# Autodesk Inventor assembly: Robotunits GUS_4041 (75)
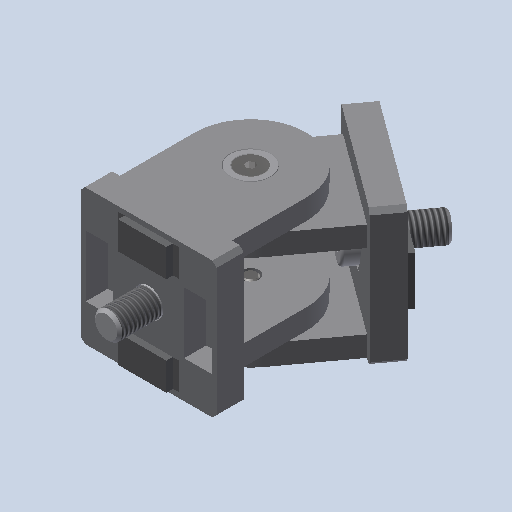
[picture p0: Inventor's stored thumbnail of the model, 512x512]
Saved by Autodesk Inventor 2023 (Build 270158000, 158)
## iProperties
Category: PARTsolutions
Company: ROBOTUNITS
Created: 2023-08-22
Part Number: Robotunits GUS_4041 (75)
Catalog Web Link: www.cadenas.de
Description: GUS 4_41-Elbow joint with clamp, kit
Vendor: ROBOTUNITS
Document SubType Name: Assembly
Designer: psAdmin
Manufacturer: ROBOTUNITS
Mass: 54.643 g
Surface Area: 289.943 cm^2
Volume: 52.1063 cm^3
Density: 1.04868 g/cm^3
PSOL_IDENT_0: {$CADENAS_DATA/23d-libs/robotunits/profil_und_verbindungstechnik/verbindungstechnik_raster_40/gus404
PSOL_IDENT_1: 1_asmtbl.prj},211 {VTYP=3D},{STYP=ASSTAB},{NB=Robotunits GUS_4041 (75)},{LINA=Robotunits GUS_4041},{
PSOL_IDENT_2: NN=GUS 4_41},{DATE=20.06.2022 09:55:41},{GEOMDATE=24.10.2014 07:53:29},{VERSION=},{LINEID=10},{WBVAR=
PSOL_IDENT_3: WINKEL},{WBNUMERIC=WINKEL}  {NB=Robotunits GUS_4041 (75)},{LINA=Robotunits GUS_4041},{KT=DUMMY},{ART
PSOL_IDENT_4: IKEL=GUS_4041},{WINKEL=75},{PPATH=parts/gus4041_sbl.prj},{FORM=1.000},{ROB=GUS4041},{ROBX=http://www
PSOL_IDENT_5: .robotunits.com/$CADENAS_LANGUAGE./Webshop/Verbindungstechnik/shopitem/gelenk-set/180/}
NB: Robotunits GUS_4041 (75)
NN: GUS 4_41
NT: Elbow joint with clamp, kit
NBSYN: Robotunits $ARTIKEL. ($WINKEL.)
LINA: Robotunits GUS_4041
CATALOG: Robotunits
ARTIKEL: GUS_4041
WINKEL: 75
ROB: GUS4041
SUPPLIER: ROBOTUNITS
ARTICLENO: Robotunits GUS_4041 (75)
BOMINFO: Robotunits GUS_4041
CREATOR: CADENAS GmbH
Title: Robotunits GUS_4041
Author: Cadenas PARTsolutions
Comments: Elbow joint with clamp, kit
## Documents named in this file (7)
- C:\work\robots\butler_2.0\body_model\parts\Elbow joint 40\Elbow joint 40.iam
- C:\work\robots\butler_2.0\body_model\parts\Elbow joint 40\Robotunits GUS_4040 75.ipt
- C:\work\robots\butler_2.0\body_model\parts\Elbow joint 40\GUS Zentriereinsatz.ipt
- C:\work\robots\butler_2.0\body_model\parts\Elbow joint 40\Robotunits IBS M8x16.ipt
- C:\work\robots\butler_2.0\body_model\parts\Elbow joint 40\Robotunits GUS_4040 -90.ipt
- C:\Users\chriboehm\Documents\Inventor\Content Center Files\R2023\en-US\DIN 7991(2)\DIN 7991 - M4x12.ipt
- C:\work\robots\butler_2.0\body_model\parts\Elbow joint 40\Washer.ipt
## Components (12 placed, 6 different names)
1. Robotunits GUS_4040 75:1 — Flush:1, Mate:7, Mate:10, Mate:13, Flush:4
2. GUS Zentriereinsatz:1
3. GUS Zentriereinsatz:2
4. Robotunits IBS M8x16:1
5. Robotunits GUS_4040 -90:1 — Mate:1, Mate:2, Mate:3, Mate:4, Mate:5, Mate:6, Flush:1, Mate:7, Mate:8, Mate:9, Mate:11, Mate:12, Flush:2
6. GUS Zentriereinsatz:3 — Mate:4, Mate:5, Mate:6
7. GUS Zentriereinsatz:4 — Mate:1, Mate:2, Mate:3
8. Robotunits IBS M8x16:2 — Mate:8, Mate:9
9. DIN 7991 M4x12:1 — Mate:10, Flush:5
10. DIN 7991 M4x12:2 — Mate:11, Flush:3
11. Washer:1 — Mate:12, Flush:2, Flush:3
12. Washer:2 — Mate:13, Flush:4, Flush:5
## Relationships (18: Mate 13, Flush 5)
- Mate:1: Robotunits GUS_4040 -90:1 ↔ GUS Zentriereinsatz:4
- Mate:2: Robotunits GUS_4040 -90:1 ↔ GUS Zentriereinsatz:4
- Mate:3: Robotunits GUS_4040 -90:1 ↔ GUS Zentriereinsatz:4
- Mate:4: Robotunits GUS_4040 -90:1 ↔ GUS Zentriereinsatz:3
- Mate:5: Robotunits GUS_4040 -90:1 ↔ GUS Zentriereinsatz:3
- Mate:6: Robotunits GUS_4040 -90:1 ↔ GUS Zentriereinsatz:3
- Flush:1: Robotunits GUS_4040 75:1 ↔ Robotunits GUS_4040 -90:1
- Mate:7: Robotunits GUS_4040 75:1 ↔ Robotunits GUS_4040 -90:1
- Mate:8: Robotunits GUS_4040 -90:1 ↔ Robotunits IBS M8x16:2
- Mate:9: Robotunits GUS_4040 -90:1 ↔ Robotunits IBS M8x16:2
- Mate:10: Robotunits GUS_4040 75:1 ↔ DIN 7991 M4x12:1
- Mate:11: Robotunits GUS_4040 -90:1 ↔ DIN 7991 M4x12:2
- Mate:12: Robotunits GUS_4040 -90:1 ↔ Washer:1
- Flush:2: Robotunits GUS_4040 -90:1 ↔ Washer:1
- Flush:3: DIN 7991 M4x12:2 ↔ Washer:1
- Mate:13: Robotunits GUS_4040 75:1 ↔ Washer:2
- Flush:4: Robotunits GUS_4040 75:1 ↔ Washer:2
- Flush:5: DIN 7991 M4x12:1 ↔ Washer:2
